# Autodesk Inventor assembly: Hepheaestes38v2 1
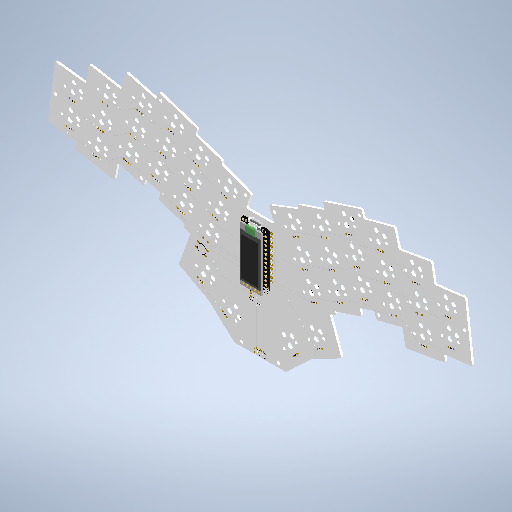
[picture p0: Inventor's stored thumbnail of the model, 512x512]
Saved by Autodesk Inventor 2025 (Build 290162000, 162)
## iProperties
Company: Kicad
Created: 2025-11-22
Part Number: Hepheaestes38v2 1
Description: KiCad electronic assembly
Document SubType Name: Assembly
Designer: User
Authority: Unknown
Sending System: KiCad to STEP converter
Preprocessor: Open CASCADE STEP processor 7.9
Title: Hepheaestes38v2.step
Author: Pcbnew
## Documents named in this file (8)
- C:\Users\User\Hephaestes38-zmk\PCB, Case\Case V2\Hepheaestes38v2 CAD\Hepheaestes38v2.iam
- C:\Users\User\Hephaestes38-zmk\PCB, Case\Case V2\Hepheaestes38v2 CAD\Hepheaestes38v2_copper.ipt
- C:\Users\User\Hephaestes38-zmk\PCB, Case\Case V2\Hepheaestes38v2 CAD\Hepheaestes38v2_pad.ipt
- C:\Users\User\Hephaestes38-zmk\PCB, Case\Case V2\Hepheaestes38v2 CAD\Hepheaestes38v2_via.ipt
- C:\Users\User\Hephaestes38-zmk\PCB, Case\Case V2\Hepheaestes38v2 CAD\Hepheaestes38v2_silkscreen.ipt
- C:\Users\User\Hephaestes38-zmk\PCB, Case\Case V2\Hepheaestes38v2 CAD\Hepheaestes38v2_PCB.ipt
- C:\Users\User\Hephaestes38-zmk\PCB, Case\Case V2\Hepheaestes38v2 CAD\Nice Nano V2.iam
- C:\Users\User\Hephaestes38-zmk\PCB, Case\Case V2\Hepheaestes38v2 CAD\nice!view\nice!view.ipt
## Components (7 placed, 7 different names)
1. 1
2. 2 — Mate:2, Mate:3, Mate:5, Mate:6
3. 3
4. 4
5. 5 — Mate:1, Mate:4
6. Nice Nano V2:1 [sub-assembly] — Mate:1, Mate:2, Mate:3
7. nice!view:1 — Mate:4, Mate:5, Mate:6
## Relationships (6: Mate 6)
- Mate:1 (2.54 mm): 5 ↔ Nice Nano V2:1
- Mate:2: 2 ↔ Nice Nano V2:1
- Mate:3: 2 ↔ Nice Nano V2:1
- Mate:4 (5.08 mm): 5 ↔ nice!view:1
- Mate:5: 2 ↔ nice!view:1
- Mate:6: 2 ↔ nice!view:1
